# Autodesk Inventor assembly: tosaerba
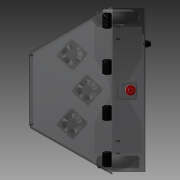
[picture p0: Inventor's stored thumbnail of the model, 180x180]
Saved by Autodesk Inventor 2014 SP2 (Build 180246200, 246)
## iProperties
Created: 2019-04-05
Part Number: tosaerba
Document SubType Name: Assembly
Designer: GauchoHP
Author: GauchoHP
## Documents named in this file (19)
- E:\Dati\Documenti_Emanuele\Svago - Varie\tosaerba\LAWNMOWER-ROBOT-from-Hoverboard-\LawnmowerMechanicalProject\3D PROJECT - INVENTOR 2014\tosaerba.iam
- E:\Dati\Documenti_Emanuele\Svago - Varie\tosaerba\LAWNMOWER-ROBOT-from-Hoverboard-\LawnmowerMechanicalProject\3D PROJECT - INVENTOR 2014\aluminium base plate\piastra.ipt
- C:\Users\GauchoHP\Desktop\old_desktop\tosaerba\LAWNMOWER-ROBOT-from-Hoverboard-\LawnmowerMechanicalProject\3D PROJECT - INVENTOR 2014\motor for blades\old\old1_multicopter_motor\motore.iam
- E:\Dati\Documenti_Emanuele\Svago - Varie\tosaerba\LAWNMOWER-ROBOT-from-Hoverboard-\LawnmowerMechanicalProject\3D PROJECT - INVENTOR 2014\rotating wheels\Assembly15.iam
- E:\Dati\Documenti_Emanuele\Svago - Varie\tosaerba\LAWNMOWER-ROBOT-from-Hoverboard-\LawnmowerMechanicalProject\3D PROJECT - INVENTOR 2014\hoverboard\hoverboard naked.iam
- E:\Dati\Documenti_Emanuele\Svago - Varie\tosaerba\LAWNMOWER-ROBOT-from-Hoverboard-\LawnmowerMechanicalProject\3D PROJECT - INVENTOR 2014\rotating wheels\Assembly1.iam
- E:\Dati\Documenti_Emanuele\Svago - Varie\tosaerba\LAWNMOWER-ROBOT-from-Hoverboard-\LawnmowerMechanicalProject\3D PROJECT - INVENTOR 2014\cover plexiglass\coverPolicarbonato2.ipt
- E:\Dati\Documenti_Emanuele\Svago - Varie\tosaerba\LAWNMOWER-ROBOT-from-Hoverboard-\LawnmowerMechanicalProject\3D PROJECT - INVENTOR 2014\cover plexiglass\sponda laterale policarbonato.ipt
- C:\Users\GauchoHP\Desktop\old_desktop\tosaerba\LAWNMOWER-ROBOT-from-Hoverboard-\LawnmowerMechanicalProject\3D PROJECT - INVENTOR 2014\blades\dadoAutobloccante.ipt
- C:\Users\GauchoHP\Desktop\old_desktop\tosaerba\LAWNMOWER-ROBOT-from-Hoverboard-\LawnmowerMechanicalProject\3D PROJECT - INVENTOR 2014\blades\vite.ipt
- C:\Users\GauchoHP\Desktop\old_desktop\tosaerba\LAWNMOWER-ROBOT-from-Hoverboard-\LawnmowerMechanicalProject\3D PROJECT - INVENTOR 2014\blades\supportoCuscinettoAlto.ipt
- C:\Users\GauchoHP\Desktop\old_desktop\tosaerba\LAWNMOWER-ROBOT-from-Hoverboard-\LawnmowerMechanicalProject\3D PROJECT - INVENTOR 2014\blades\bearing.ipt
- C:\Users\GauchoHP\Desktop\old_desktop\tosaerba\LAWNMOWER-ROBOT-from-Hoverboard-\LawnmowerMechanicalProject\3D PROJECT - INVENTOR 2014\blades\bladeSupport.ipt
- C:\Users\GauchoHP\Desktop\old_desktop\tosaerba\LAWNMOWER-ROBOT-from-Hoverboard-\LawnmowerMechanicalProject\3D PROJECT - INVENTOR 2014\blades\boltCap.ipt
- C:\Users\GauchoHP\Desktop\old_desktop\tosaerba\LAWNMOWER-ROBOT-from-Hoverboard-\LawnmowerMechanicalProject\3D PROJECT - INVENTOR 2014\blades\lametta.ipt
- E:\Dati\Documenti_Emanuele\Svago - Varie\tosaerba\LAWNMOWER-ROBOT-from-Hoverboard-\LawnmowerMechanicalProject\3D PROJECT - INVENTOR 2014\sensors\SensorAssembly.iam
- E:\Dati\Documenti_Emanuele\Svago - Varie\tosaerba\LAWNMOWER-ROBOT-from-Hoverboard-\LawnmowerMechanicalProject\3D PROJECT - INVENTOR 2014\emergency stop button\Emergency Stop Button - Ass.ipt
- E:\Dati\Documenti_Emanuele\Svago - Varie\tosaerba\LAWNMOWER-ROBOT-from-Hoverboard-\LawnmowerMechanicalProject\3D PROJECT - INVENTOR 2014\power button\powerButtonAssembly.iam
- E:\Dati\Documenti_Emanuele\Svago - Varie\tosaerba\LAWNMOWER-ROBOT-from-Hoverboard-\LawnmowerMechanicalProject\3D PROJECT - INVENTOR 2014\motor with blades\motorWithBlades.iam
## Components (30 placed, 18 different names)
1. piastra:1 — Mate:8, Mate:37, Mate:45, Mate:46, Flush:3, Mate:47, Flush:4, Mate:48, Mate:49, Flush:5, Flush:6, Flush:7, Flush:8, Mate:50, Mate:51, Mate:52, Mate:54, Mate:55, Mate:81, Mate:82, Flush:14, Mate:110, Flush:25, Angle:1, Mate:111, Mate:114, Angle:3, Angle:4
2. motore:1 [sub-assembly] — Mate:8, Mate:84, Flush:14
3. Assembly15:1 [sub-assembly] — Mate:54, Mate:55
4. hoverboard naked:1 [sub-assembly] — Mate:37, Flush:2, Mate:48, Mate:112, Mate:115
5. Assembly1:1 [sub-assembly] — Mate:51, Mate:52
6. coverPolicarbonato2:1 — Flush:2, Mate:45, Mate:46, Flush:4, Mate:85, Mate:86, Mate:87, Mate:88, Flush:15, Mate:89, Mate:90, Mate:94, Mate:97, Flush:16, Flush:23, Flush:24, Mate:106, Mate:107, Mate:108, Mate:109
7. sponda laterale policarbonato:1 — Mate:49, Flush:5, Flush:6
8. sponda laterale policarbonato:2 — Flush:7, Flush:8, Mate:50
9. dadoAutobloccante:1 — Mate:65, Flush:10, Mate:67
10. dadoAutobloccante:2 — Mate:68, Mate:71, Mate:82
11. vite:1 — Mate:61, Mate:62, Mate:63, Mate:65, Mate:66, Mate:68, Mate:69, Mate:83, Mate:84
12. supportoCuscinettoAlto:1 — Mate:57, Flush:9, Mate:63, Mate:64
13. bearing:1 — Mate:57, Flush:9, Mate:62, Mate:83
14. bearing:2 — Mate:59, Mate:60
15. supportoCuscinettoAlto:2 — Mate:59, Mate:60, Mate:61, Mate:64, Flush:10, Mate:81
16. bladeSupport:1 — Mate:66, Mate:67, Mate:70, Mate:72, Mate:73, Mate:74, Flush:11, Mate:75, Mate:76, Flush:12, Mate:77, Mate:78, Flush:13, Mate:79, Mate:80
17. boltCap:1 — Mate:69, Mate:70, Mate:71
18. lametta:1 — Mate:72, Mate:73, Mate:74
19. lametta:2 — Flush:11, Mate:75, Mate:76
20. lametta:3 — Flush:12, Mate:77, Mate:78
21. lametta:4 — Flush:13, Mate:79, Mate:80
22. SensorAssembly:1 [sub-assembly] — Mate:85, Flush:15, Mate:89, Flush:18
23. SensorAssembly:2 [sub-assembly] — Mate:86, Mate:94, Flush:17
24. SensorAssembly:3 [sub-assembly] — Mate:87, Mate:97, Flush:16, Flush:17
25. SensorAssembly:4 [sub-assembly] — Mate:88, Mate:90, Flush:18
26. Emergency Stop Button - Ass:1 — Flush:23, Flush:24, Mate:106
27. powerButtonAssembly:1 [sub-assembly] — Mate:107, Mate:108, Mate:109
28. motorWithBlades:1 [sub-assembly] — Mate:110, Flush:25, Angle:1, Mate:116, Mate:117
29. motorWithBlades:2 [sub-assembly] — Mate:114, Angle:3, Mate:115, Mate:116
30. motorWithBlades:3 [sub-assembly] — Mate:111, Mate:112, Angle:4, Mate:117
## Relationships (81: Mate 58, Flush 20, Angle 3)
- Mate:8: piastra:1 ↔ motore:1
- Mate:37: piastra:1 ↔ hoverboard naked:1
- Flush:2 (5.5 mm): hoverboard naked:1 ↔ coverPolicarbonato2:1
- Mate:45: piastra:1 ↔ coverPolicarbonato2:1
- Mate:46 (20 mm): piastra:1 ↔ coverPolicarbonato2:1
- Flush:3: piastra:1
- Mate:47 (66 mm): piastra:1
- Flush:4 (8 mm): piastra:1 ↔ coverPolicarbonato2:1
- Mate:48 (5 mm): piastra:1 ↔ hoverboard naked:1
- Mate:49: piastra:1 ↔ sponda laterale policarbonato:1
- Flush:5: piastra:1 ↔ sponda laterale policarbonato:1
- Flush:6 (20 mm): piastra:1 ↔ sponda laterale policarbonato:1
- Flush:7: piastra:1 ↔ sponda laterale policarbonato:2
- Flush:8 (-20 mm): piastra:1 ↔ sponda laterale policarbonato:2
- Mate:50: piastra:1 ↔ sponda laterale policarbonato:2
- Mate:51: piastra:1 ↔ Assembly1:1
- Mate:52: piastra:1 ↔ Assembly1:1
- Mate:54: piastra:1 ↔ Assembly15:1
- Mate:55: piastra:1 ↔ Assembly15:1
- Mate:57: supportoCuscinettoAlto:1 ↔ bearing:1
- Mate:59: bearing:2 ↔ supportoCuscinettoAlto:2
- Mate:60: bearing:2 ↔ supportoCuscinettoAlto:2
- Mate:61: vite:1 ↔ supportoCuscinettoAlto:2
- Flush:9: supportoCuscinettoAlto:1 ↔ bearing:1
- Mate:62: vite:1 ↔ bearing:1
- Mate:63 (-3 mm): vite:1 ↔ supportoCuscinettoAlto:1
- Mate:64 (3 mm): supportoCuscinettoAlto:1 ↔ supportoCuscinettoAlto:2
- Mate:65: dadoAutobloccante:1 ↔ vite:1
- Flush:10 (-10 mm): dadoAutobloccante:1 ↔ supportoCuscinettoAlto:2
- Mate:66: vite:1 ↔ bladeSupport:1
- Mate:67: dadoAutobloccante:1 ↔ bladeSupport:1
- Mate:68: dadoAutobloccante:2 ↔ vite:1
- Mate:69: vite:1 ↔ boltCap:1
- Mate:70: bladeSupport:1 ↔ boltCap:1
- Mate:71: dadoAutobloccante:2 ↔ boltCap:1
- Mate:72: bladeSupport:1 ↔ lametta:1
- Mate:73: bladeSupport:1 ↔ lametta:1
- Mate:74: bladeSupport:1 ↔ lametta:1
- Flush:11 (-0.8 mm): bladeSupport:1 ↔ lametta:2
- Mate:75: bladeSupport:1 ↔ lametta:2
- Mate:76: bladeSupport:1 ↔ lametta:2
- Flush:12 (-0.8 mm): bladeSupport:1 ↔ lametta:3
- Mate:77: bladeSupport:1 ↔ lametta:3
- Mate:78: bladeSupport:1 ↔ lametta:3
- Flush:13 (-0.8 mm): bladeSupport:1 ↔ lametta:4
- Mate:79: bladeSupport:1 ↔ lametta:4
- Mate:80: bladeSupport:1 ↔ lametta:4
- Mate:81: piastra:1 ↔ supportoCuscinettoAlto:2
- Mate:82: piastra:1 ↔ dadoAutobloccante:2
- Mate:83: vite:1 ↔ bearing:1
- Mate:84: motore:1 ↔ vite:1
- Flush:14 (15.364 mm): piastra:1 ↔ motore:1
- Mate:85: coverPolicarbonato2:1 ↔ SensorAssembly:1
- Mate:86: coverPolicarbonato2:1 ↔ SensorAssembly:2
- Mate:87: coverPolicarbonato2:1 ↔ SensorAssembly:3
- Mate:88: coverPolicarbonato2:1 ↔ SensorAssembly:4
- Flush:15 (20 mm): coverPolicarbonato2:1 ↔ SensorAssembly:1
- Mate:89 (3 mm): coverPolicarbonato2:1 ↔ SensorAssembly:1
- Mate:90 (3 mm): coverPolicarbonato2:1 ↔ SensorAssembly:4
- Mate:94 (3 mm): coverPolicarbonato2:1 ↔ SensorAssembly:2
- Mate:97 (3 mm): coverPolicarbonato2:1 ↔ SensorAssembly:3
- Flush:16 (20 mm): coverPolicarbonato2:1 ↔ SensorAssembly:3
- Flush:17 (167.5 mm): SensorAssembly:2 ↔ SensorAssembly:3
- Flush:18 (167.5 mm): SensorAssembly:1 ↔ SensorAssembly:4
- Flush:23 (3 mm): coverPolicarbonato2:1 ↔ Emergency Stop Button - Ass:1
- Flush:24 (-264 mm): coverPolicarbonato2:1 ↔ Emergency Stop Button - Ass:1
- Mate:106 (30 mm): coverPolicarbonato2:1 ↔ Emergency Stop Button - Ass:1
- Mate:107: coverPolicarbonato2:1 ↔ powerButtonAssembly:1
- Mate:108 (-130 mm): coverPolicarbonato2:1 ↔ powerButtonAssembly:1
- Mate:109 (-60 mm): coverPolicarbonato2:1 ↔ powerButtonAssembly:1
- Mate:110: piastra:1 ↔ motorWithBlades:1
- Flush:25 (3 mm): piastra:1 ↔ motorWithBlades:1
- Angle:1 (45 deg): piastra:1 ↔ motorWithBlades:1
- Mate:111: piastra:1 ↔ motorWithBlades:3
- Mate:112 (80 mm): hoverboard naked:1 ↔ motorWithBlades:3
- Mate:114: piastra:1 ↔ motorWithBlades:2
- Angle:3 (45 deg): piastra:1 ↔ motorWithBlades:2
- Mate:115 (80 mm): hoverboard naked:1 ↔ motorWithBlades:2
- Mate:116 (45 mm): motorWithBlades:1 ↔ motorWithBlades:2
- Angle:4 (45 deg): piastra:1 ↔ motorWithBlades:3
- Mate:117 (45 mm): motorWithBlades:1 ↔ motorWithBlades:3
